# Autodesk Inventor assembly: フランジ
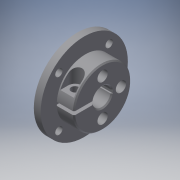
[picture p0: Inventor's stored thumbnail of the model, 180x180]
Saved by Autodesk Inventor 2019 (Build 230136000, 136)
## iProperties
Created: 2020-10-25
Part Number: フランジ
Material: 一般
Document SubType Name: Assembly
Designer: zhept
Author: zhept
## iProperties of the stored document SCS0808CP3.iam
Company: CADENAS
Created: 2020-10-25
Part Number: SCS0808CP3
Material: 一般
Description: STEP AP203
Document SubType Name: Assembly
Designer: zhept
Sending System: PARTsolutions
Title: p:/temp/worker_8/temp/exporttempdir_1868_723_K7orS/format_0/SCS0808CP3.stp
Author: License CC BY-ND 4.0
Revision Number: NONE
## iProperties of the stored document _SCS  0808CP3-part.ipt
Created: 2020-09-25
Part Number: _SCS  0808CP3-part
Material: 一般
Document SubType Name: Modeling
Designer: zhept
Density: 1 g/cm^3
Appearance: 既定
Author: zhept
Revision Number: NONE
## Documents named in this file (5)
- C:\Users\zhept\OneDrive\大学\rrst\足回り2020\フランジ.iam
- C:\Users\zhept\OneDrive\大学\rrst\足回り2020\フランジ.ipt
- **C:\Users\zhept\OneDrive\大学\rrst\足回り2020\フランジ.iam*LocalDocs*xIseyrzuaBz0wuhksVkwozee2Yh*SCS0808CP3.iam
- C:\Users\zhept\OneDrive\大学\rrst\足回り2020\IWATA_SCS0808CP3\SCS0808CP3.stp
- **C:\Users\zhept\OneDrive\大学\rrst\足回り2020\フランジ.iam*LocalDocs*xKmahfw4bRqgdetot13k3sopqHg*_SCS  0808CP3-part.ipt
## Components (2 placed, 2 different names)
1. フランジ:1 — 挿入:1, 挿入:2
2. SCS0808CP3:1 [sub-assembly] — 挿入:1, 挿入:2
## Relationships (2: Insert 2)
- 挿入:1 [Insert]: フランジ:1 ↔ SCS0808CP3:1
- 挿入:2 [Insert]: フランジ:1 ↔ SCS0808CP3:1
